# Autodesk Inventor assembly: Assembly5
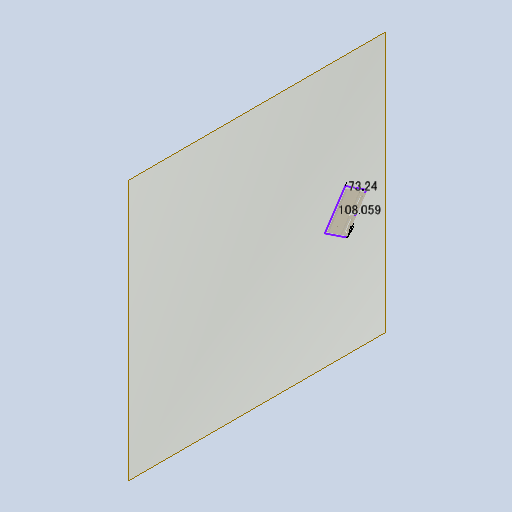
[picture p0: Inventor's stored thumbnail of the model, 512x512]
Saved by Autodesk Inventor 2025.2 (Build 292293000, 293)
## iProperties
Created: 2024-12-17
Part Number: Assembly5
Document SubType Name: Assembly
Designer: haruy
Author: haruy
## Documents named in this file (3)
- C:\Users\haruy\Documents\ロボコン\NHK2025\cad\cnc\Assembly5.iam
- C:\Users\haruy\Documents\ロボコン\NHK2025\cad\nagahisa\belt_liner\belt_liner_v1_Plate_1.ipt
- C:\Users\haruy\Documents\ロボコン\NHK2025\cad\nagahisa\belt_liner\belt_liner_v1_Plate_9.ipt
## Components (3 placed, 2 different names)
1. belt_liner_v1_Plate_1:1 — フラッシュ:1, フラッシュ:4, メイト:1, メイト:2
2. belt_liner_v1_Plate_9:1 — フラッシュ:2, フラッシュ:4, メイト:1
3. belt_liner_v1_Plate_9:2 — フラッシュ:3, メイト:2
## Relationships (6: Flush 4, Mate 2)
- フラッシュ:1 [Flush]: belt_liner_v1_Plate_1:1
- フラッシュ:2 [Flush]: belt_liner_v1_Plate_9:1
- フラッシュ:3 [Flush]: belt_liner_v1_Plate_9:2
- フラッシュ:4 [Flush]: belt_liner_v1_Plate_1:1 ↔ belt_liner_v1_Plate_9:1
- メイト:1 [Mate] (5 mm): belt_liner_v1_Plate_1:1 ↔ belt_liner_v1_Plate_9:1
- メイト:2 [Mate] (5 mm): belt_liner_v1_Plate_1:1 ↔ belt_liner_v1_Plate_9:2
